# Autodesk Inventor assembly: 104.001.01_Foerderband_GBG
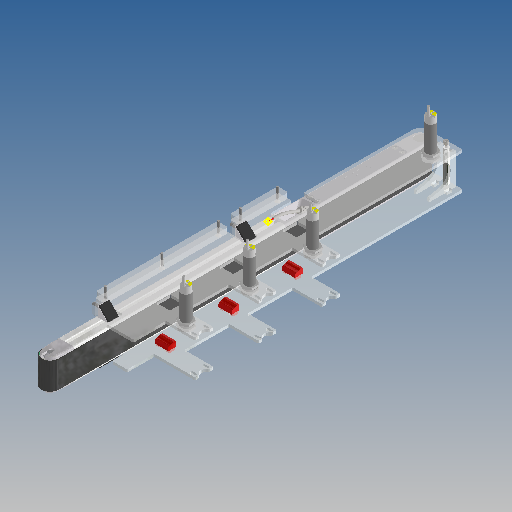
[picture p0: Inventor's stored thumbnail of the model, 512x512]
Saved by Autodesk Inventor 2021 (Build 250183000, 183)
## iProperties
Created: 2021-11-21
Part Number: 104.001.01_Foerderband_GBG
Document SubType Name: Assembly
Designer: Oliver Ungerer
Author: Oliver Ungerer
## Documents named in this file (17)
- E:\Dokumente\MCI-Mechatronik\Master\Semester_3\Projekt_2_Neu\105_Foerderbandeinheit\205.001.01_ZB_Foerderbandeinheit.iam
- E:\Dokumente\MCI-Mechatronik\Master\Semester_3\Projekt_2_Neu\105_Foerderbandeinheit\505.005.01_Foerderband.ipt
- E:\Dokumente\MCI-Mechatronik\Master\Semester_3\Projekt_2_Neu\105_Foerderbandeinheit\205.003.01_ZB_ITEM_Winkelsatz_5_20x20.iam
- E:\Dokumente\MCI-Mechatronik\Master\Semester_3\Projekt_2_Neu\105_Foerderbandeinheit\105.004.01_Auflageplatte_FB.ipt
- E:\Dokumente\MCI-Mechatronik\Master\Semester_3\Projekt_2_Neu\104_Extrudereinheit\Schrauben\DIN EN ISO 4762 - M5 x 12.ipt
- E:\Dokumente\MCI-Mechatronik\Master\Semester_3\Projekt_2_Neu\105_Foerderbandeinheit\105.005.01_Endanschlag_Flasche.ipt
- E:\Dokumente\MCI-Mechatronik\Master\Semester_3\Projekt_2_Neu\105_Foerderbandeinheit\105.001.01_Wand_Foerderband.ipt
- E:\Dokumente\MCI-Mechatronik\Master\Semester_3\Projekt_2_Neu\105_Foerderbandeinheit\105.005.01_Foerderband_Halterung_hinten.ipt
- E:\Dokumente\MCI-Mechatronik\Master\Semester_3\Projekt_2_Neu\105_Foerderbandeinheit\105.006.01_Distanzbuchse.ipt
- E:\Dokumente\MCI-Mechatronik\Master\Semester_3\Projekt_2_Neu\105_Foerderbandeinheit\105.002.01_Distanz_Wand.ipt
- E:\Dokumente\MCI-Mechatronik\Master\Semester_3\Projekt_2_Neu\105_Foerderbandeinheit\105.003.01_Distanz_Wand.ipt
- E:\Dokumente\MCI-Mechatronik\Master\Semester_3\Projekt_2_Neu\105_Foerderbandeinheit\Schrauben\DIN_EN_ISO_10642_M4x25.ipt
- E:\Dokumente\MCI-Mechatronik\Master\Semester_3\Projekt_2_Neu\105_Foerderbandeinheit\Schrauben\DIN_EN_ISO_4762_M5x20.ipt
- E:\Dokumente\MCI-Mechatronik\Master\Semester_3\Projekt_2_Neu\105_Foerderbandeinheit\105.007.01_Positionsausgleich_Stopper.ipt
- E:\Dokumente\MCI-Mechatronik\Master\Semester_3\Projekt_2_Neu\105_Foerderbandeinheit\Schrauben\DIN_912_M3x8.ipt
- E:\Dokumente\MCI-Mechatronik\Master\Semester_3\Projekt_2_Neu\105_Foerderbandeinheit\505.006.01_BALLUFF-BCS-M18BBN1-PSC80D-EP021.ipt
- E:\Dokumente\MCI-Mechatronik\Master\Semester_3\Projekt_2_Neu\105_Foerderbandeinheit\505.007.01_Nut_M18x1.ipt
## Components (52 placed, 16 different names)
1. 505.005.01_Foerderband:1 — Passend:1, Passend:2, Winkel:1, Passend:3, Winkel:2, Passend:4, Passend:5, Passend:6, Winkel:3, Passend:7, Passend:8, Winkel:4, Passend:11, Passend:14, Passend:17, Passend:20, Passend:25, Passend:26, Fluchtend:15, Passend:60
2. 205.003.01_ZB_ITEM_Winkelsatz_5_20x20:1 [sub-assembly] — Passend:1, Passend:2, Winkel:1, Passend:9, Fluchtend:1, Fluchtend:2, Fluchtend:13, Passend:27, Passend:67, Passend:68
3. 205.003.01_ZB_ITEM_Winkelsatz_5_20x20:2 [sub-assembly] — Passend:3, Winkel:2, Passend:4, Passend:12, Fluchtend:6, Fluchtend:14, Passend:69, Passend:70
4. 205.003.01_ZB_ITEM_Winkelsatz_5_20x20:3 [sub-assembly] — Passend:7, Passend:8, Winkel:4, Passend:18, Fluchtend:12, Fluchtend:13, Passend:21, Passend:25, Passend:73, Passend:74
5. 205.003.01_ZB_ITEM_Winkelsatz_5_20x20:4 [sub-assembly] — Passend:5, Passend:6, Winkel:3, Passend:15, Fluchtend:9, Fluchtend:14, Passend:21, Passend:61, Passend:71, Passend:72
6. 105.004.01_Auflageplatte_FB:1 — Passend:10, Fluchtend:2, Fluchtend:3
7. 105.004.01_Auflageplatte_FB:2 — Passend:9, Passend:10, Fluchtend:1, Passend:11, Fluchtend:3
8. 105.004.01_Auflageplatte_FB:3 — Passend:12, Passend:13, Fluchtend:4, Fluchtend:5, Fluchtend:6
9. 105.004.01_Auflageplatte_FB:4 — Passend:13, Fluchtend:4, Fluchtend:5, Passend:14
10. 105.004.01_Auflageplatte_FB:5 — Passend:15, Passend:16, Fluchtend:7, Fluchtend:8, Fluchtend:9, Passend:17
11. 105.004.01_Auflageplatte_FB:6 — Passend:18, Passend:19, Fluchtend:10, Fluchtend:11, Fluchtend:12, Passend:20
12. 105.004.01_Auflageplatte_FB:7 — Passend:19, Fluchtend:10, Fluchtend:11
13. 105.004.01_Auflageplatte_FB:8 — Passend:16, Fluchtend:7, Fluchtend:8
14. DIN EN ISO 4762 - M5 x 12:1 — Passend:30, Passend:31
15. DIN EN ISO 4762 - M5 x 12:2 — Passend:28, Passend:29
16. DIN EN ISO 4762 - M5 x 12:3 — Passend:32, Passend:33
17. 105.005.01_Foerderband_Halterung_hinten:1 — Passend:26, Passend:27, Fluchtend:15, Passend:28, Passend:29, Passend:30, Passend:31, Passend:32, Passend:33, Passend:48, Passend:50, Passend:51, Fluchtend:16, Passend:75, Passend:76, Passend:77, Passend:84, Passend:85, Passend:86
18. 105.005.01_Endanschlag_Flasche:1
19. 105.005.01_Endanschlag_Flasche:2
20. 105.001.01_Wand_Foerderband:1 — Passend:49, Passend:52, Passend:53, Passend:54, Passend:55, Passend:56, Passend:57, Passend:58, Passend:59, Passend:60, Passend:61, Fluchtend:16, Passend:62, Passend:63, Passend:64, Passend:65, Passend:66, Fluchtend:17, Fluchtend:18, Fluchtend:19, Fluchtend:20, Fluchtend:21, Passend:78, Passend:79, Passend:80, Passend:87, Passend:88, Passend:89, Passend:90, Fluchtend:22, Passend:99, Passend:100, Passend:101, Passend:102, Fluchtend:23, Passend:103, Passend:104, Fluchtend:24, Passend:105, Passend:106, Fluchtend:25, Passend:107, Passend:108, Passend:109
21. 105.006.01_Distanzbuchse:1 — Passend:48, Passend:49
22. DIN EN ISO 4762 - M5 x 12:4 — Passend:52, Passend:53
23. DIN EN ISO 4762 - M5 x 12:5 — Passend:50, Passend:51
24. 105.002.01_Distanz_Wand:1 — Passend:55, Passend:58, Passend:59
25. 105.003.01_Distanz_Wand:1 — Passend:54, Passend:56, Passend:57
26. DIN_EN_ISO_10642_M4x25:1 — Passend:62, Fluchtend:21
27. DIN_EN_ISO_10642_M4x25:2 — Passend:63, Fluchtend:20
28. DIN_EN_ISO_10642_M4x25:3 — Passend:64, Fluchtend:19
29. DIN_EN_ISO_10642_M4x25:4 — Passend:66, Fluchtend:17
30. DIN_EN_ISO_10642_M4x25:5 — Passend:65, Fluchtend:18
31. DIN_EN_ISO_4762_M5x20:1 — Passend:67, Passend:68
32. DIN_EN_ISO_4762_M5x20:2 — Passend:69, Passend:70
33. DIN_EN_ISO_4762_M5x20:3 — Passend:73, Passend:74
34. DIN_EN_ISO_4762_M5x20:4 — Passend:71, Passend:72
35. 105.007.01_Positionsausgleich_Stopper:1 — Passend:75, Passend:78, Passend:81, Passend:107
36. 105.007.01_Positionsausgleich_Stopper:2 — Passend:76, Passend:79, Passend:82, Passend:108
37. 105.007.01_Positionsausgleich_Stopper:3 — Passend:77, Passend:80, Passend:83, Passend:109
38. DIN_912_M3x8:1 — Passend:81, Passend:84
39. DIN_912_M3x8:2 — Passend:82, Passend:85
40. DIN_912_M3x8:3 — Passend:83, Passend:86
41. 505.006.01_BALLUFF-BCS-M18BBN1-PSC80D-EP021:1 — Passend:87, Passend:97, Passend:98, Fluchtend:22
42. 505.006.01_BALLUFF-BCS-M18BBN1-PSC80D-EP021:2 — Passend:88, Passend:95, Passend:96, Fluchtend:23
43. 505.006.01_BALLUFF-BCS-M18BBN1-PSC80D-EP021:3 — Passend:89, Passend:93, Passend:94, Fluchtend:24
44. 505.006.01_BALLUFF-BCS-M18BBN1-PSC80D-EP021:4 — Passend:90, Passend:91, Passend:92, Fluchtend:25
45. 505.007.01_Nut_M18x1:1 — Passend:98, Passend:100
46. 505.007.01_Nut_M18x1:2 — Passend:97, Passend:99
47. 505.007.01_Nut_M18x1:3 — Passend:96, Passend:102
48. 505.007.01_Nut_M18x1:4 — Passend:95, Passend:101
49. 505.007.01_Nut_M18x1:5 — Passend:94, Passend:104
50. 505.007.01_Nut_M18x1:6 — Passend:93, Passend:103
51. 505.007.01_Nut_M18x1:7 — Passend:92, Passend:106
52. 505.007.01_Nut_M18x1:8 — Passend:91, Passend:105
## Relationships (127: Mate 98, Flush 25, Angle 4)
- Passend:1 [Mate]: 505.005.01_Foerderband:1 ↔ 205.003.01_ZB_ITEM_Winkelsatz_5_20x20:1
- Passend:2 [Mate] (-15 mm): 505.005.01_Foerderband:1 ↔ 205.003.01_ZB_ITEM_Winkelsatz_5_20x20:1
- Winkel:1 [Angle] (270 deg): 505.005.01_Foerderband:1 ↔ 205.003.01_ZB_ITEM_Winkelsatz_5_20x20:1
- Passend:3 [Mate]: 505.005.01_Foerderband:1 ↔ 205.003.01_ZB_ITEM_Winkelsatz_5_20x20:2
- Winkel:2 [Angle] (270 deg): 505.005.01_Foerderband:1 ↔ 205.003.01_ZB_ITEM_Winkelsatz_5_20x20:2
- Passend:4 [Mate] (-15 mm): 505.005.01_Foerderband:1 ↔ 205.003.01_ZB_ITEM_Winkelsatz_5_20x20:2
- Passend:5 [Mate]: 505.005.01_Foerderband:1 ↔ 205.003.01_ZB_ITEM_Winkelsatz_5_20x20:4
- Passend:6 [Mate] (-15 mm): 505.005.01_Foerderband:1 ↔ 205.003.01_ZB_ITEM_Winkelsatz_5_20x20:4
- Winkel:3 [Angle] (90 deg): 505.005.01_Foerderband:1 ↔ 205.003.01_ZB_ITEM_Winkelsatz_5_20x20:4
- Passend:7 [Mate]: 505.005.01_Foerderband:1 ↔ 205.003.01_ZB_ITEM_Winkelsatz_5_20x20:3
- Passend:8 [Mate] (-15 mm): 505.005.01_Foerderband:1 ↔ 205.003.01_ZB_ITEM_Winkelsatz_5_20x20:3
- Winkel:4 [Angle] (90 deg): 505.005.01_Foerderband:1 ↔ 205.003.01_ZB_ITEM_Winkelsatz_5_20x20:3
- Passend:9 [Mate]: 205.003.01_ZB_ITEM_Winkelsatz_5_20x20:1 ↔ 105.004.01_Auflageplatte_FB:2
- Passend:10 [Mate]: 105.004.01_Auflageplatte_FB:1 ↔ 105.004.01_Auflageplatte_FB:2
- Fluchtend:1 [Flush]: 205.003.01_ZB_ITEM_Winkelsatz_5_20x20:1 ↔ 105.004.01_Auflageplatte_FB:2
- Fluchtend:2 [Flush]: 205.003.01_ZB_ITEM_Winkelsatz_5_20x20:1 ↔ 105.004.01_Auflageplatte_FB:1
- Passend:11 [Mate]: 505.005.01_Foerderband:1 ↔ 105.004.01_Auflageplatte_FB:2
- Fluchtend:3 [Flush]: 105.004.01_Auflageplatte_FB:1 ↔ 105.004.01_Auflageplatte_FB:2
- Passend:12 [Mate]: 205.003.01_ZB_ITEM_Winkelsatz_5_20x20:2 ↔ 105.004.01_Auflageplatte_FB:3
- Passend:13 [Mate]: 105.004.01_Auflageplatte_FB:3 ↔ 105.004.01_Auflageplatte_FB:4
- Fluchtend:4 [Flush]: 105.004.01_Auflageplatte_FB:3 ↔ 105.004.01_Auflageplatte_FB:4
- Fluchtend:5 [Flush]: 105.004.01_Auflageplatte_FB:3 ↔ 105.004.01_Auflageplatte_FB:4
- Fluchtend:6 [Flush]: 205.003.01_ZB_ITEM_Winkelsatz_5_20x20:2 ↔ 105.004.01_Auflageplatte_FB:3
- Passend:14 [Mate]: 505.005.01_Foerderband:1 ↔ 105.004.01_Auflageplatte_FB:4
- Passend:15 [Mate]: 205.003.01_ZB_ITEM_Winkelsatz_5_20x20:4 ↔ 105.004.01_Auflageplatte_FB:5
- Passend:16 [Mate]: 105.004.01_Auflageplatte_FB:5 ↔ 105.004.01_Auflageplatte_FB:8
- Fluchtend:7 [Flush]: 105.004.01_Auflageplatte_FB:5 ↔ 105.004.01_Auflageplatte_FB:8
- Fluchtend:8 [Flush]: 105.004.01_Auflageplatte_FB:5 ↔ 105.004.01_Auflageplatte_FB:8
- Fluchtend:9 [Flush]: 205.003.01_ZB_ITEM_Winkelsatz_5_20x20:4 ↔ 105.004.01_Auflageplatte_FB:5
- Passend:17 [Mate]: 505.005.01_Foerderband:1 ↔ 105.004.01_Auflageplatte_FB:5
- Passend:18 [Mate]: 205.003.01_ZB_ITEM_Winkelsatz_5_20x20:3 ↔ 105.004.01_Auflageplatte_FB:6
- Passend:19 [Mate]: 105.004.01_Auflageplatte_FB:6 ↔ 105.004.01_Auflageplatte_FB:7
- Fluchtend:10 [Flush]: 105.004.01_Auflageplatte_FB:6 ↔ 105.004.01_Auflageplatte_FB:7
- Fluchtend:11 [Flush]: 105.004.01_Auflageplatte_FB:6 ↔ 105.004.01_Auflageplatte_FB:7
- Fluchtend:12 [Flush]: 205.003.01_ZB_ITEM_Winkelsatz_5_20x20:3 ↔ 105.004.01_Auflageplatte_FB:6
- Passend:20 [Mate]: 505.005.01_Foerderband:1 ↔ 105.004.01_Auflageplatte_FB:6
- Fluchtend:13 [Flush]: 205.003.01_ZB_ITEM_Winkelsatz_5_20x20:1 ↔ 205.003.01_ZB_ITEM_Winkelsatz_5_20x20:3
- Fluchtend:14 [Flush]: 205.003.01_ZB_ITEM_Winkelsatz_5_20x20:2 ↔ 205.003.01_ZB_ITEM_Winkelsatz_5_20x20:4
- Passend:21 [Mate] (240 mm): 205.003.01_ZB_ITEM_Winkelsatz_5_20x20:3 ↔ 205.003.01_ZB_ITEM_Winkelsatz_5_20x20:4
- Passend:25 [Mate] (100 mm): 505.005.01_Foerderband:1 ↔ 205.003.01_ZB_ITEM_Winkelsatz_5_20x20:3
- Passend:26 [Mate]: 505.005.01_Foerderband:1 ↔ 105.005.01_Foerderband_Halterung_hinten:1
- Passend:27 [Mate] (5 mm): 205.003.01_ZB_ITEM_Winkelsatz_5_20x20:1 ↔ 105.005.01_Foerderband_Halterung_hinten:1
- Fluchtend:15 [Flush]: 505.005.01_Foerderband:1 ↔ 105.005.01_Foerderband_Halterung_hinten:1
- Passend:28 [Mate]: DIN EN ISO 4762 - M5 x 12:2 ↔ 105.005.01_Foerderband_Halterung_hinten:1
- Passend:29 [Mate]: DIN EN ISO 4762 - M5 x 12:2 ↔ 105.005.01_Foerderband_Halterung_hinten:1
- Passend:30 [Mate]: DIN EN ISO 4762 - M5 x 12:1 ↔ 105.005.01_Foerderband_Halterung_hinten:1
- Passend:31 [Mate]: DIN EN ISO 4762 - M5 x 12:1 ↔ 105.005.01_Foerderband_Halterung_hinten:1
- Passend:32 [Mate]: DIN EN ISO 4762 - M5 x 12:3 ↔ 105.005.01_Foerderband_Halterung_hinten:1
- Passend:33 [Mate]: DIN EN ISO 4762 - M5 x 12:3 ↔ 105.005.01_Foerderband_Halterung_hinten:1
- [Mate]: 105.005.01_Foerderband_Halterung_hinten:1 ↔ 105.005.01_Endanschlag_Flasche:1
- [Mate]: 105.005.01_Foerderband_Halterung_hinten:1 ↔ 105.005.01_Endanschlag_Flasche:1
- [Mate]: 105.005.01_Foerderband_Halterung_hinten:1 ↔ 105.005.01_Endanschlag_Flasche:2
- [Mate]: 105.005.01_Foerderband_Halterung_hinten:1 ↔ 105.005.01_Endanschlag_Flasche:2
- [Mate]: 105.005.01_Foerderband_Halterung_hinten:1 ↔ 105.005.01_Endanschlag_Flasche:2
- [Mate]: 105.005.01_Endanschlag_Flasche:1 ↔ 105.001.01_Wand_Foerderband:1
- Passend:48 [Mate]: 105.005.01_Foerderband_Halterung_hinten:1 ↔ 105.006.01_Distanzbuchse:1
- Passend:49 [Mate]: 105.001.01_Wand_Foerderband:1 ↔ 105.006.01_Distanzbuchse:1
- Passend:50 [Mate]: 105.005.01_Foerderband_Halterung_hinten:1 ↔ DIN EN ISO 4762 - M5 x 12:5
- Passend:51 [Mate]: 105.005.01_Foerderband_Halterung_hinten:1 ↔ DIN EN ISO 4762 - M5 x 12:5
- Passend:52 [Mate]: 105.001.01_Wand_Foerderband:1 ↔ DIN EN ISO 4762 - M5 x 12:4
- Passend:53 [Mate]: 105.001.01_Wand_Foerderband:1 ↔ DIN EN ISO 4762 - M5 x 12:4
- Passend:54 [Mate]: 105.001.01_Wand_Foerderband:1 ↔ 105.003.01_Distanz_Wand:1
- Passend:55 [Mate]: 105.001.01_Wand_Foerderband:1 ↔ 105.002.01_Distanz_Wand:1
- Passend:56 [Mate]: 105.001.01_Wand_Foerderband:1 ↔ 105.003.01_Distanz_Wand:1
- Passend:57 [Mate]: 105.001.01_Wand_Foerderband:1 ↔ 105.003.01_Distanz_Wand:1
- Passend:58 [Mate]: 105.001.01_Wand_Foerderband:1 ↔ 105.002.01_Distanz_Wand:1
- Passend:59 [Mate]: 105.001.01_Wand_Foerderband:1 ↔ 105.002.01_Distanz_Wand:1
- Passend:60 [Mate]: 505.005.01_Foerderband:1 ↔ 105.001.01_Wand_Foerderband:1
- Passend:61 [Mate] (1 mm): 205.003.01_ZB_ITEM_Winkelsatz_5_20x20:4 ↔ 105.001.01_Wand_Foerderband:1
- Fluchtend:16 [Flush]: 105.005.01_Foerderband_Halterung_hinten:1 ↔ 105.001.01_Wand_Foerderband:1
- Passend:62 [Mate]: 105.001.01_Wand_Foerderband:1 ↔ DIN_EN_ISO_10642_M4x25:1
- Passend:63 [Mate]: 105.001.01_Wand_Foerderband:1 ↔ DIN_EN_ISO_10642_M4x25:2
- Passend:64 [Mate]: 105.001.01_Wand_Foerderband:1 ↔ DIN_EN_ISO_10642_M4x25:3
- Passend:65 [Mate]: 105.001.01_Wand_Foerderband:1 ↔ DIN_EN_ISO_10642_M4x25:5
- Passend:66 [Mate]: 105.001.01_Wand_Foerderband:1 ↔ DIN_EN_ISO_10642_M4x25:4
- Fluchtend:17 [Flush]: 105.001.01_Wand_Foerderband:1 ↔ DIN_EN_ISO_10642_M4x25:4
- Fluchtend:18 [Flush]: 105.001.01_Wand_Foerderband:1 ↔ DIN_EN_ISO_10642_M4x25:5
- Fluchtend:19 [Flush]: 105.001.01_Wand_Foerderband:1 ↔ DIN_EN_ISO_10642_M4x25:3
- Fluchtend:20 [Flush]: 105.001.01_Wand_Foerderband:1 ↔ DIN_EN_ISO_10642_M4x25:2
- Fluchtend:21 [Flush]: 105.001.01_Wand_Foerderband:1 ↔ DIN_EN_ISO_10642_M4x25:1
- Passend:67 [Mate]: 205.003.01_ZB_ITEM_Winkelsatz_5_20x20:1 ↔ DIN_EN_ISO_4762_M5x20:1
- Passend:68 [Mate]: 205.003.01_ZB_ITEM_Winkelsatz_5_20x20:1 ↔ DIN_EN_ISO_4762_M5x20:1
- Passend:69 [Mate]: 205.003.01_ZB_ITEM_Winkelsatz_5_20x20:2 ↔ DIN_EN_ISO_4762_M5x20:2
- Passend:70 [Mate]: 205.003.01_ZB_ITEM_Winkelsatz_5_20x20:2 ↔ DIN_EN_ISO_4762_M5x20:2
- Passend:71 [Mate]: 205.003.01_ZB_ITEM_Winkelsatz_5_20x20:4 ↔ DIN_EN_ISO_4762_M5x20:4
- Passend:72 [Mate]: 205.003.01_ZB_ITEM_Winkelsatz_5_20x20:4 ↔ DIN_EN_ISO_4762_M5x20:4
- Passend:73 [Mate]: 205.003.01_ZB_ITEM_Winkelsatz_5_20x20:3 ↔ DIN_EN_ISO_4762_M5x20:3
- Passend:74 [Mate]: 205.003.01_ZB_ITEM_Winkelsatz_5_20x20:3 ↔ DIN_EN_ISO_4762_M5x20:3
- Passend:75 [Mate]: 105.005.01_Foerderband_Halterung_hinten:1 ↔ 105.007.01_Positionsausgleich_Stopper:1
- Passend:76 [Mate]: 105.005.01_Foerderband_Halterung_hinten:1 ↔ 105.007.01_Positionsausgleich_Stopper:2
- Passend:77 [Mate]: 105.005.01_Foerderband_Halterung_hinten:1 ↔ 105.007.01_Positionsausgleich_Stopper:3
- Passend:78 [Mate]: 105.001.01_Wand_Foerderband:1 ↔ 105.007.01_Positionsausgleich_Stopper:1
- Passend:79 [Mate]: 105.001.01_Wand_Foerderband:1 ↔ 105.007.01_Positionsausgleich_Stopper:2
- Passend:80 [Mate]: 105.001.01_Wand_Foerderband:1 ↔ 105.007.01_Positionsausgleich_Stopper:3
- Passend:81 [Mate]: 105.007.01_Positionsausgleich_Stopper:1 ↔ DIN_912_M3x8:1
- Passend:82 [Mate]: 105.007.01_Positionsausgleich_Stopper:2 ↔ DIN_912_M3x8:2
- Passend:83 [Mate]: 105.007.01_Positionsausgleich_Stopper:3 ↔ DIN_912_M3x8:3
- Passend:84 [Mate]: 105.005.01_Foerderband_Halterung_hinten:1 ↔ DIN_912_M3x8:1
- Passend:85 [Mate]: 105.005.01_Foerderband_Halterung_hinten:1 ↔ DIN_912_M3x8:2
- Passend:86 [Mate]: 105.005.01_Foerderband_Halterung_hinten:1 ↔ DIN_912_M3x8:3
- Passend:87 [Mate] (-4 mm): 105.001.01_Wand_Foerderband:1 ↔ 505.006.01_BALLUFF-BCS-M18BBN1-PSC80D-EP021:1
- Passend:88 [Mate] (-4 mm): 105.001.01_Wand_Foerderband:1 ↔ 505.006.01_BALLUFF-BCS-M18BBN1-PSC80D-EP021:2
- Passend:89 [Mate] (-4 mm): 105.001.01_Wand_Foerderband:1 ↔ 505.006.01_BALLUFF-BCS-M18BBN1-PSC80D-EP021:3
- Passend:90 [Mate]: 105.001.01_Wand_Foerderband:1 ↔ 505.006.01_BALLUFF-BCS-M18BBN1-PSC80D-EP021:4
- Passend:91 [Mate]: 505.006.01_BALLUFF-BCS-M18BBN1-PSC80D-EP021:4 ↔ 505.007.01_Nut_M18x1:8
- Passend:92 [Mate]: 505.006.01_BALLUFF-BCS-M18BBN1-PSC80D-EP021:4 ↔ 505.007.01_Nut_M18x1:7
- Passend:93 [Mate]: 505.006.01_BALLUFF-BCS-M18BBN1-PSC80D-EP021:3 ↔ 505.007.01_Nut_M18x1:6
- Passend:94 [Mate]: 505.006.01_BALLUFF-BCS-M18BBN1-PSC80D-EP021:3 ↔ 505.007.01_Nut_M18x1:5
- Passend:95 [Mate]: 505.006.01_BALLUFF-BCS-M18BBN1-PSC80D-EP021:2 ↔ 505.007.01_Nut_M18x1:4
- Passend:96 [Mate]: 505.006.01_BALLUFF-BCS-M18BBN1-PSC80D-EP021:2 ↔ 505.007.01_Nut_M18x1:3
- Passend:97 [Mate]: 505.006.01_BALLUFF-BCS-M18BBN1-PSC80D-EP021:1 ↔ 505.007.01_Nut_M18x1:2
- Passend:98 [Mate]: 505.006.01_BALLUFF-BCS-M18BBN1-PSC80D-EP021:1 ↔ 505.007.01_Nut_M18x1:1
- Fluchtend:22 [Flush] (-6 mm): 105.001.01_Wand_Foerderband:1 ↔ 505.006.01_BALLUFF-BCS-M18BBN1-PSC80D-EP021:1
- Passend:99 [Mate]: 105.001.01_Wand_Foerderband:1 ↔ 505.007.01_Nut_M18x1:2
- Passend:100 [Mate]: 105.001.01_Wand_Foerderband:1 ↔ 505.007.01_Nut_M18x1:1
- Passend:101 [Mate]: 105.001.01_Wand_Foerderband:1 ↔ 505.007.01_Nut_M18x1:4
- Passend:102 [Mate]: 105.001.01_Wand_Foerderband:1 ↔ 505.007.01_Nut_M18x1:3
- Fluchtend:23 [Flush] (-6 mm): 105.001.01_Wand_Foerderband:1 ↔ 505.006.01_BALLUFF-BCS-M18BBN1-PSC80D-EP021:2
- Passend:103 [Mate]: 105.001.01_Wand_Foerderband:1 ↔ 505.007.01_Nut_M18x1:6
- Passend:104 [Mate]: 105.001.01_Wand_Foerderband:1 ↔ 505.007.01_Nut_M18x1:5
- Fluchtend:24 [Flush] (-6 mm): 105.001.01_Wand_Foerderband:1 ↔ 505.006.01_BALLUFF-BCS-M18BBN1-PSC80D-EP021:3
- Passend:105 [Mate]: 105.001.01_Wand_Foerderband:1 ↔ 505.007.01_Nut_M18x1:8
- Passend:106 [Mate]: 105.001.01_Wand_Foerderband:1 ↔ 505.007.01_Nut_M18x1:7
- Fluchtend:25 [Flush] (-4 mm): 105.001.01_Wand_Foerderband:1 ↔ 505.006.01_BALLUFF-BCS-M18BBN1-PSC80D-EP021:4
- Passend:107 [Mate] (-17.5 mm): 105.001.01_Wand_Foerderband:1 ↔ 105.007.01_Positionsausgleich_Stopper:1
- Passend:108 [Mate] (-17.5 mm): 105.001.01_Wand_Foerderband:1 ↔ 105.007.01_Positionsausgleich_Stopper:2
- Passend:109 [Mate] (-17.5 mm): 105.001.01_Wand_Foerderband:1 ↔ 105.007.01_Positionsausgleich_Stopper:3
